# Autodesk Inventor assembly: Montagem3
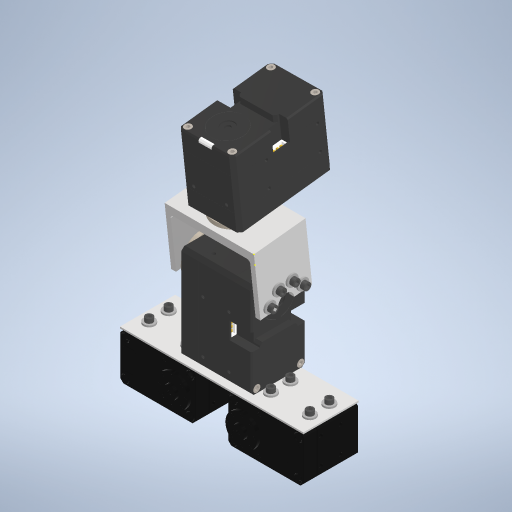
[picture p0: Inventor's stored thumbnail of the model, 512x512]
Saved by Autodesk Inventor 2024 (Build 280153000, 153)
## iProperties
Created: 2024-10-14
Part Number: Montagem3
Document SubType Name: Assembly
Designer: robof
Author: robof
## Documents named in this file (5)
- C:\Github_mecanica\Artigo\componentes\Montagem3.iam
- C:\Github_mecanica\Artigo\componentes\Dynamixel_XM540.ipt
- C:\Github_mecanica\Artigo\componentes\linkzinho_motor.ipt
- C:\Github_mecanica\Artigo\componentes\chapinha_garra.ipt
- C:\Github_mecanica\Artigo\componentes\XM430-W350-R.ipt
## Components (6 placed, 4 different names)
1. chapinha_garra:1 — Alinhado:1, Coincidente:1, Coincidente:2, Coincidente:3, Alinhado:2, Alinhado:3, Coincidente:4, Alinhado:4, Alinhado:5, Coincidente:5, Coincidente:6, Coincidente:7
2. XM430-W350-R:1 — Coincidente:4, Alinhado:4, Alinhado:5
3. XM430-W350-R:2 — Coincidente:3, Alinhado:2, Alinhado:3
4. Dynamixel_XM540:1 — Coincidente:5, Coincidente:6, Coincidente:7, Coincidente:8, Coincidente:9
5. linkzinho_motor:1 — Coincidente:8, Coincidente:9, Coincidente:10, Coincidente:11
6. Dynamixel_XM540:2 — Coincidente:10, Coincidente:11
## Relationships (16: Mate 11, Flush 5)
- Alinhado:1 [Flush]: chapinha_garra:1
- Coincidente:1 [Mate]: chapinha_garra:1
- Coincidente:2 [Mate]: chapinha_garra:1
- Coincidente:3 [Mate]: chapinha_garra:1 ↔ XM430-W350-R:2
- Alinhado:2 [Flush]: chapinha_garra:1 ↔ XM430-W350-R:2
- Alinhado:3 [Flush]: chapinha_garra:1 ↔ XM430-W350-R:2
- Coincidente:4 [Mate]: chapinha_garra:1 ↔ XM430-W350-R:1
- Alinhado:4 [Flush]: chapinha_garra:1 ↔ XM430-W350-R:1
- Alinhado:5 [Flush]: chapinha_garra:1 ↔ XM430-W350-R:1
- Coincidente:5 [Mate]: chapinha_garra:1 ↔ Dynamixel_XM540:1
- Coincidente:6 [Mate]: chapinha_garra:1 ↔ Dynamixel_XM540:1
- Coincidente:7 [Mate] (34.5 mm): chapinha_garra:1 ↔ Dynamixel_XM540:1
- Coincidente:8 [Mate]: Dynamixel_XM540:1 ↔ linkzinho_motor:1
- Coincidente:9 [Mate]: Dynamixel_XM540:1 ↔ linkzinho_motor:1
- Coincidente:10 [Mate]: linkzinho_motor:1 ↔ Dynamixel_XM540:2
- Coincidente:11 [Mate]: linkzinho_motor:1 ↔ Dynamixel_XM540:2
